# Autodesk Inventor assembly: robot1
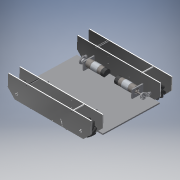
[picture p0: Inventor's stored thumbnail of the model, 180x180]
Saved by Autodesk Inventor 2019 (Build 230136000, 136)
## iProperties
Created: 2020-10-03
Part Number: robot1
Document SubType Name: Assembly
Designer: User
Author: User
## Documents named in this file (3)
- C:\Robotics\CAD\2020-21-CAD\main robot\robot1.iam
- C:\Robotics\CAD\2020-21-CAD\main robot\main plate.ipt
- C:\Robotics\CAD\2020-21-CAD\Drivetrain\InvertedDriveTrain.iam
## Components (3 placed, 2 different names)
1. main plate:1 — Mate:1, Mate:2, Flush:1, Mate:3, Mate:4, Flush:2
2. InvertedDriveTrain:1 [sub-assembly] — Mate:1, Mate:2, Flush:1
3. InvertedDriveTrain:2 [sub-assembly] — Mate:3, Mate:4, Flush:2
## Relationships (6: Mate 4, Flush 2)
- Mate:1: main plate:1 ↔ InvertedDriveTrain:1
- Mate:2: main plate:1 ↔ InvertedDriveTrain:1
- Flush:1: main plate:1 ↔ InvertedDriveTrain:1
- Mate:3: main plate:1 ↔ InvertedDriveTrain:2
- Mate:4: main plate:1 ↔ InvertedDriveTrain:2
- Flush:2: main plate:1 ↔ InvertedDriveTrain:2
